# Autodesk Inventor assembly: hotend mount
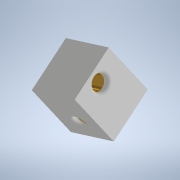
[picture p0: Inventor's stored thumbnail of the model, 180x180]
Saved by Autodesk Inventor 2020.4 (Build 244396000, 396)
## iProperties
Created: 2021-03-19
Part Number: hotend mount
Document SubType Name: Assembly
Designer: AOB
Mass: 70.4266 g
Surface Area: 130.626 cm^2
Volume: 26.3058 cm^3
Density: 2.67722 g/cm^3
Author: AOB
## Documents named in this file (3)
- C:\Users\marti\Documents\Inventor\ProjectBoron\Boron Ultima\hotend mount.iam
- C:\Users\marti\Documents\Inventor\ProjectBoron\Boron Ultima\lm8uu-graphite.ipt
- C:\Users\marti\Documents\Inventor\ProjectBoron\Boron Ultima\hotend mount.ipt
## Components (4 placed, 2 different names)
1. hotend mount:1 — Flush:2, Rigid:1, Mate:1, Mate:3, Mate:4
2. hotend mount:2 — Flush:2, Rigid:1, Mate:2
3. lm8uu-graphite:1 — Mate:3, Mate:4
4. lm8uu-graphite:2 — Mate:1, Mate:2
## Relationships (6: Mate 4, Flush 1, WeldJoint 1)
- Flush:2: hotend mount:1 ↔ hotend mount:2
- Rigid:1 [WeldJoint]: hotend mount:1 ↔ hotend mount:2
- Mate:1: hotend mount:1 ↔ lm8uu-graphite:2
- Mate:2: hotend mount:2 ↔ lm8uu-graphite:2
- Mate:3: hotend mount:1 ↔ lm8uu-graphite:1
- Mate:4: hotend mount:1 ↔ lm8uu-graphite:1
